# Autodesk Inventor assembly: サイクロイド減速機
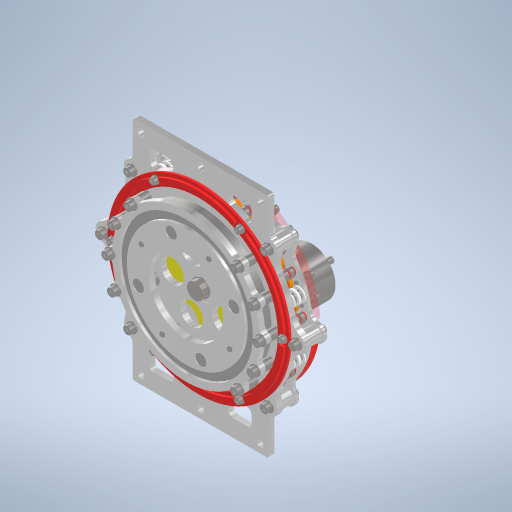
[picture p0: Inventor's stored thumbnail of the model, 512x512]
Saved by Autodesk Inventor 2024 (Build 280153000, 153)
## iProperties
Created: 2023-05-29
Part Number: サイクロイド減速機
Document SubType Name: Assembly
Designer: yuta2
Mass: 2238.9 g
Surface Area: 3502.49 cm^2
Volume: 607.759 cm^3
Density: 3.68387 g/cm^3
Author: yuta2
## Documents named in this file (32)
- C:\Users\yuta2\Documents\Inventor\CycloidDrive\サイクロイド減速機_大型\サイクロイド減速機.iam
- C:\Users\yuta2\Documents\Inventor\CycloidDrive\サイクロイド減速機_大型\サイクロイド減速機パラメータ.ipt
- C:\Users\yuta2\Documents\Inventor\CycloidDrive\サイクロイド減速機_大型\サイクロイドギア.ipt
- C:\Users\yuta2\Documents\Inventor\CycloidDrive\サイクロイド減速機_大型\ベース板_出力側.ipt
- C:\Users\yuta2\Documents\Inventor\CycloidDrive\サイクロイド減速機_大型\偏心軸ユニット.iam
- C:\Users\yuta2\Documents\Inventor\CycloidDrive\サイクロイド減速機_大型\出力板ユニット.iam
- C:\Users\yuta2\Documents\Inventor\CycloidDrive\サイクロイド減速機_大型\入力軸.ipt
- C:\Users\yuta2\Documents\Inventor\CycloidDrive\サイクロイド減速機_大型\出力ベアリング抑え.ipt
- C:\Users\yuta2\Documents\Inventor\CycloidDrive\サイクロイド減速機_大型\サイクロイド減速機\デザイン アクセラレータ\ボルト締結1.iam
- C:\Users\yuta2\Documents\Inventor\CycloidDrive\サイクロイド減速機_大型\外周ピンユニット.iam
- C:\Users\yuta2\Documents\Inventor\CycloidDrive\サイクロイド減速機_大型\ベース板入力側.ipt
- C:\Users\yuta2\Documents\Inventor\CycloidDrive\ベアリング\SMF148ZZ.ipt
- C:\Users\yuta2\Documents\Inventor\CycloidDrive\サイクロイド減速機_大型\RZ735.ipt
- C:\Users\yuta2\Documents\Inventor\CycloidDrive\サイクロイド減速機_大型\サイクロイド減速機\デザイン アクセラレータ\平歯車1.iam
- C:\Users\yuta2\Documents\Inventor\CycloidDrive\サイクロイド減速機_大型\サイクロイド減速機\デザイン アクセラレータ\平歯車2.iam
- C:\Users\yuta2\Documents\Inventor\CycloidDrive\サイクロイド減速機_大型\モーターマウント板.ipt
- C:\Users\yuta2\Documents\Inventor\CycloidDrive\サイクロイド減速機_大型\モーターマウント板固定部品.ipt
- C:\Users\yuta2\Documents\Inventor\CycloidDrive\サイクロイド減速機_大型\モーターマウント板固定部品2.ipt
- C:\Users\yuta2\Documents\Inventor\CycloidDrive\共通部品\インサートナットM4.ipt
- C:\Users\yuta2\Documents\Inventor\CycloidDrive\サイクロイド減速機_大型\サイクロイド減速機\デザイン アクセラレータ\ボルト締結2.iam
- C:\Users\yuta2\Documents\Inventor\CycloidDrive\サイクロイド減速機_大型\サイクロイド減速機\デザイン アクセラレータ\ボルト締結3.iam
- C:\Users\yuta2\Documents\Inventor\CycloidDrive\サイクロイド減速機_大型\外周ピン抑え.ipt
- C:\Users\yuta2\Documents\Inventor\CycloidDrive\サイクロイド減速機_大型\サイクロイド減速機\デザイン アクセラレータ\ボルト締結4.iam
- C:\Users\yuta2\Documents\Inventor\CycloidDrive\サイクロイド減速機_大型\ベース板連結棒.ipt
- C:\Users\yuta2\Documents\Inventor\CycloidDrive\サイクロイド減速機_大型\サイクロイド減速機\デザイン アクセラレータ\ボルト締結5.iam
- C:\Users\yuta2\Documents\Inventor\CycloidDrive\サイクロイド減速機_大型\出力ベアリング固定スペーサ.ipt
- C:\Users\yuta2\Documents\Inventor\CycloidDrive\サイクロイド減速機_大型\セットカラーSSCCJ8-5.ipt
- C:\Users\yuta2\Documents\Inventor\CycloidDrive\サイクロイド減速機_大型\ギアスペーサ1.ipt
- C:\Users\yuta2\Documents\Inventor\CycloidDrive\サイクロイド減速機_大型\ギアスペーサ2.ipt
- C:\Users\yuta2\Documents\Inventor\CycloidDrive\サイクロイド減速機_大型\外周ベアリングスペーサ1.ipt
- C:\Users\yuta2\Documents\Inventor\CycloidDrive\サイクロイド減速機_大型\外周ベアリングスペーサ.ipt
- C:\Users\yuta2\Documents\Inventor\CycloidDrive\サイクロイド減速機_大型\入力駆動ギアスペーサ.ipt
## Components (185 placed, 26 different names)
1. サイクロイド減速機パラメータ:1
2. サイクロイドギア:1 — 回転:1, 正接:5
3. ベース板_出力側:1 — 回転:3, 回転:9, 回転:25, 回転:26, 回転:30, メイト:18, メイト:19
4. 偏心軸ユニット:1 [sub-assembly] — 回転:1, 回転:2, 回転:5, 回転:10
5. サイクロイドギア:2 — 回転:2, 正接:2, 正接:4
6. 出力板ユニット:1 [sub-assembly] — 回転:3, 回転:5, 回転:6, 回転:32, 正接:4, 正接:5
7. 入力軸:1 — 回転:33, 回転:36, 回転:37
8. 出力ベアリング抑え:1 — 回転:6, メイト:15, メイト:16, 回転:29
9. ボルト締結:1 [sub-assembly] — メイト:15, メイト:16
10. ベース板入力側:1 — 円柱状:1, 回転:10, 回転:13, 回転:17, 回転:24, メイト:6, 回転:27, 回転:34, メイト:17
11. RZ735:1 — 回転:14, 回転:15, 回転:16
12. 平歯車:1 [sub-assembly] — 回転:13, 回転:47
13. 平歯車:2 [sub-assembly] — 回転:14
14. モーターマウント板:1 — 回転:15, 回転:16, 回転:18, 回転:19, 回転:20, 回転:21, メイト:13, メイト:14, 回転:35
15. モーターマウント板固定部品:1 — 回転:17, 回転:18, 回転:19, 回転:22, 回転:24, メイト:5
16. モーターマウント板固定部品2:1 — 回転:20, 回転:21, 回転:23
17. ボルト締結:2 [sub-assembly] — メイト:13, メイト:14
18. ボルト締結:3 [sub-assembly] — メイト:5, メイト:6
19. 外周ピン抑え:1 — 回転:25, 回転:26, メイト:7, メイト:8
20. SMF148ZZ:2 — 回転:35
21. SMF148ZZ:3 — 回転:32, 回転:33
22. SMF148ZZ:4 — 回転:34
23. セットカラーSSCCJ8-5:1 — 回転:36
24. セットカラーSSCCJ8-5:2 — 回転:37
25. 入力駆動ギアスペーサ:1 — 回転:47
26. 外周ピンユニット:1 [sub-assembly] — 回転:9, 円柱状:1
27. 外周ピンユニット:2 [sub-assembly]
28. 外周ピンユニット:3 [sub-assembly]
29. 外周ピンユニット:4 [sub-assembly]
30. 外周ピンユニット:5 [sub-assembly]
31. 外周ピンユニット:6 [sub-assembly]
32. 外周ピンユニット:7 [sub-assembly]
33. 外周ピンユニット:8 [sub-assembly]
34. 外周ピンユニット:9 [sub-assembly]
35. 外周ピンユニット:10 [sub-assembly] — 正接:2
36. 外周ピンユニット:11 [sub-assembly]
37. 外周ピンユニット:12 [sub-assembly]
38. 外周ピンユニット:13 [sub-assembly]
39. 外周ピンユニット:14 [sub-assembly]
40. 外周ピンユニット:15 [sub-assembly]
41. 外周ピンユニット:16 [sub-assembly]
42. 外周ピンユニット:17 [sub-assembly]
43. 外周ピンユニット:18 [sub-assembly]
44. 外周ピンユニット:19 [sub-assembly]
45. 外周ピンユニット:20 [sub-assembly]
46. 外周ピンユニット:21 [sub-assembly]
47. 外周ピンユニット:22 [sub-assembly] — メイト:17, 回転:38, 回転:39, 回転:40
48. 外周ピンユニット:23 [sub-assembly]
49. 外周ピンユニット:24 [sub-assembly]
50. 外周ピンユニット:25 [sub-assembly]
51. 外周ピンユニット:26 [sub-assembly] — 回転:42, 回転:43, 回転:46
52. 外周ピンユニット:27 [sub-assembly] — 回転:41, 回転:44, 回転:45
53. 外周ピンユニット:28 [sub-assembly]
54. 外周ピンユニット:29 [sub-assembly]
55. 外周ピンユニット:30 [sub-assembly]
56. インサートナットM4:1 — 回転:22
57. インサートナットM4:3
58. インサートナットM4:4
59. インサートナットM4:5
60. インサートナットM4:6
61. インサートナットM4:7
62. インサートナットM4:2 — 回転:23
63. インサートナットM4:8
64. インサートナットM4:9
65. インサートナットM4:10
66. インサートナットM4:11
67. インサートナットM4:12
68. ボルト締結:4 [sub-assembly] — メイト:7, メイト:8
69. ボルト締結:5 [sub-assembly]
70. ボルト締結:6 [sub-assembly]
71. ボルト締結:7 [sub-assembly]
72. ボルト締結:8 [sub-assembly]
73. ボルト締結:9 [sub-assembly]
74. 外周ベアリングスペーサ1:4 — 回転:44
75. 外周ベアリングスペーサ:1 — 回転:45
76. 外周ベアリングスペーサ1:1 — 回転:41
77. 外周ベアリングスペーサ1:3 — 回転:43
78. 外周ベアリングスペーサ:2 — 回転:46
79. 外周ベアリングスペーサ1:2 — 回転:42
80. ギアスペーサ1:2 — 回転:39
81. ギアスペーサ2:1 — 回転:40
82. ギアスペーサ1:1 — 回転:38
83. 外周ベアリングスペーサ1:5
84. 外周ベアリングスペーサ:3
85. 外周ベアリングスペーサ1:6
86. 外周ベアリングスペーサ1:7
87. 外周ベアリングスペーサ:4
88. 外周ベアリングスペーサ1:8
89. ギアスペーサ1:3
90. ギアスペーサ2:2
91. ギアスペーサ1:4
92. 外周ベアリングスペーサ1:9
93. 外周ベアリングスペーサ:5
94. 外周ベアリングスペーサ1:10
95. 外周ベアリングスペーサ1:11
96. 外周ベアリングスペーサ:6
97. 外周ベアリングスペーサ1:12
98. ギアスペーサ1:5
99. ギアスペーサ2:3
100. ギアスペーサ1:6
101. 外周ベアリングスペーサ1:13
102. 外周ベアリングスペーサ:7
103. 外周ベアリングスペーサ1:14
104. 外周ベアリングスペーサ1:15
105. 外周ベアリングスペーサ:8
106. 外周ベアリングスペーサ1:16
107. ギアスペーサ1:7
108. ギアスペーサ2:4
109. ギアスペーサ1:8
110. 外周ベアリングスペーサ1:17
111. 外周ベアリングスペーサ:9
112. 外周ベアリングスペーサ1:18
113. 外周ベアリングスペーサ1:19
114. 外周ベアリングスペーサ:10
115. 外周ベアリングスペーサ1:20
116. ギアスペーサ1:9
117. ギアスペーサ2:5
118. ギアスペーサ1:10
119. 外周ベアリングスペーサ1:21
120. 外周ベアリングスペーサ:11
121. 外周ベアリングスペーサ1:22
122. 外周ベアリングスペーサ1:23
123. 外周ベアリングスペーサ:12
124. 外周ベアリングスペーサ1:24
125. ギアスペーサ1:11
126. ギアスペーサ2:6
127. ギアスペーサ1:12
128. 外周ベアリングスペーサ1:25
129. 外周ベアリングスペーサ:13
130. 外周ベアリングスペーサ1:26
131. 外周ベアリングスペーサ1:27
132. 外周ベアリングスペーサ:14
133. 外周ベアリングスペーサ1:28
134. ギアスペーサ1:13
135. ギアスペーサ2:7
136. ギアスペーサ1:14
137. 外周ベアリングスペーサ1:29
138. 外周ベアリングスペーサ:15
139. 外周ベアリングスペーサ1:30
140. 外周ベアリングスペーサ1:31
141. 外周ベアリングスペーサ:16
142. 外周ベアリングスペーサ1:32
143. ギアスペーサ1:15
144. ギアスペーサ2:8
145. ギアスペーサ1:16
146. 外周ベアリングスペーサ1:33
147. 外周ベアリングスペーサ:17
148. 外周ベアリングスペーサ1:34
149. 外周ベアリングスペーサ1:35
150. 外周ベアリングスペーサ:18
151. 外周ベアリングスペーサ1:36
152. ギアスペーサ1:17
153. ギアスペーサ2:9
154. ギアスペーサ1:18
155. 外周ベアリングスペーサ1:37
156. 外周ベアリングスペーサ:19
157. 外周ベアリングスペーサ1:38
158. 外周ベアリングスペーサ1:39
159. 外周ベアリングスペーサ:20
160. 外周ベアリングスペーサ1:40
161. ギアスペーサ1:19
162. ギアスペーサ2:10
163. ギアスペーサ1:20
164. ベース板連結棒:1 — 回転:27
165. ベース板連結棒:2
166. ベース板連結棒:3
167. ベース板連結棒:4
168. ベース板連結棒:5
169. ベース板連結棒:6
170. ボルト締結:10 [sub-assembly] — メイト:18, メイト:19
171. ボルト締結:11 [sub-assembly]
172. ボルト締結:12 [sub-assembly]
173. ボルト締結:13 [sub-assembly]
174. ボルト締結:14 [sub-assembly]
175. ボルト締結:15 [sub-assembly]
176. 出力ベアリング固定スペーサ:1 — 回転:29, 回転:30
177. 出力ベアリング固定スペーサ:2
178. 出力ベアリング固定スペーサ:3
179. 出力ベアリング固定スペーサ:4
180. 出力ベアリング固定スペーサ:5
181. 出力ベアリング固定スペーサ:6
182. 出力ベアリング固定スペーサ:7
183. 出力ベアリング固定スペーサ:8
184. 出力ベアリング固定スペーサ:9
185. 出力ベアリング固定スペーサ:10
## Component patterns: (30 elements, first: 外周ピンユニット:1), (6 elements, first: インサートナットM4:1), (6 elements, first: インサートナットM4:2), (6 elements, first: ボルト締結:4), (2 elements), (3 elements), (2 elements), (10 elements, first: 外周ベアリングスペーサ1:4 + 外周ベアリングスペーサ:1 + 外周ベアリングスペーサ1:1 + 外周ベアリングスペーサ1:3 + 外周ベアリングスペーサ:2 + 外周ベアリングスペーサ1:2 + ギアスペーサ1:2 + ギアスペーサ2:1 + ギアスペーサ1:1), (3 elements, first: ベース板連結棒:1), コンポーネント パターン 7:2 (3 elements), (2 elements, first: ボルト締結:10), コンポーネント パターン 9:2 (2 elements), コンポーネント パターン 9:3 (2 elements), (5 elements, first: 出力ベアリング固定スペーサ:1), コンポーネント パターン 11:2 (5 elements)
## Relationships (55: RevoluteJoint 40, Mate 11, Tangent 3, CylindricalJoint 1)
- 回転:1 [RevoluteJoint]: サイクロイドギア:1 ↔ 偏心軸ユニット:1
- 回転:2 [RevoluteJoint]: 偏心軸ユニット:1 ↔ サイクロイドギア:2
- 回転:3 [RevoluteJoint]: ベース板_出力側:1 ↔ 出力板ユニット:1
- 回転:5 [RevoluteJoint] (0.5 mm): 偏心軸ユニット:1 ↔ 出力板ユニット:1
- 回転:6 [RevoluteJoint]: 出力板ユニット:1 ↔ 出力ベアリング抑え:1
- 回転:9 [RevoluteJoint]: ベース板_出力側:1 ↔ 外周ピンユニット:1
- 円柱状:1 [CylindricalJoint]: ベース板入力側:1 ↔ 外周ピンユニット:1
- 回転:10 [RevoluteJoint] (-0.5 mm): 偏心軸ユニット:1 ↔ ベース板入力側:1
- 回転:13 [RevoluteJoint] (1 mm): ベース板入力側:1 ↔ 平歯車:1
- 回転:14 [RevoluteJoint] (0.5 mm): RZ735:1 ↔ 平歯車:2
- 回転:15 [RevoluteJoint]: RZ735:1 ↔ モーターマウント板:1
- 回転:16 [RevoluteJoint]: RZ735:1 ↔ モーターマウント板:1
- 回転:17 [RevoluteJoint]: ベース板入力側:1 ↔ モーターマウント板固定部品:1
- 回転:18 [RevoluteJoint]: モーターマウント板:1 ↔ モーターマウント板固定部品:1
- 回転:19 [RevoluteJoint]: モーターマウント板:1 ↔ モーターマウント板固定部品:1
- 回転:20 [RevoluteJoint]: モーターマウント板:1 ↔ モーターマウント板固定部品2:1
- 回転:21 [RevoluteJoint]: モーターマウント板:1 ↔ モーターマウント板固定部品2:1
- 回転:22 [RevoluteJoint]: モーターマウント板固定部品:1 ↔ インサートナットM4:1
- 回転:23 [RevoluteJoint]: モーターマウント板固定部品2:1 ↔ インサートナットM4:2
- 回転:24 [RevoluteJoint]: ベース板入力側:1 ↔ モーターマウント板固定部品:1
- メイト:5 [Mate]: モーターマウント板固定部品:1 ↔ ボルト締結:3
- メイト:6 [Mate]: ベース板入力側:1 ↔ ボルト締結:3
- 回転:25 [RevoluteJoint]: ベース板_出力側:1 ↔ 外周ピン抑え:1
- 回転:26 [RevoluteJoint]: ベース板_出力側:1 ↔ 外周ピン抑え:1
- メイト:7 [Mate]: 外周ピン抑え:1 ↔ ボルト締結:4
- メイト:8 [Mate]: 外周ピン抑え:1 ↔ ボルト締結:4
- 回転:27 [RevoluteJoint]: ベース板入力側:1 ↔ ベース板連結棒:1
- メイト:13 [Mate]: モーターマウント板:1 ↔ ボルト締結:2
- メイト:14 [Mate]: モーターマウント板:1 ↔ ボルト締結:2
- メイト:15 [Mate]: 出力ベアリング抑え:1 ↔ ボルト締結:1
- メイト:16 [Mate]: 出力ベアリング抑え:1 ↔ ボルト締結:1
- 回転:29 [RevoluteJoint]: 出力ベアリング抑え:1 ↔ 出力ベアリング固定スペーサ:1
- 回転:30 [RevoluteJoint]: ベース板_出力側:1 ↔ 出力ベアリング固定スペーサ:1
- 回転:32 [RevoluteJoint]: 出力板ユニット:1 ↔ SMF148ZZ:3
- 回転:33 [RevoluteJoint] (5 mm): 入力軸:1 ↔ SMF148ZZ:3
- 回転:34 [RevoluteJoint]: ベース板入力側:1 ↔ SMF148ZZ:4
- 回転:35 [RevoluteJoint]: モーターマウント板:1 ↔ SMF148ZZ:2
- メイト:17 [Mate]: ベース板入力側:1 ↔ 外周ピンユニット:22
- 正接:2 [Tangent]: サイクロイドギア:2 ↔ 外周ピンユニット:10
- 正接:4 [Tangent]: サイクロイドギア:2 ↔ 出力板ユニット:1
- 正接:5 [Tangent]: サイクロイドギア:1 ↔ 出力板ユニット:1
- 回転:36 [RevoluteJoint]: 入力軸:1 ↔ セットカラーSSCCJ8-5:1
- 回転:37 [RevoluteJoint]: 入力軸:1 ↔ セットカラーSSCCJ8-5:2
- メイト:18 [Mate]: ベース板_出力側:1 ↔ ボルト締結:10
- メイト:19 [Mate]: ベース板_出力側:1 ↔ ボルト締結:10
- 回転:38 [RevoluteJoint]: 外周ピンユニット:22 ↔ ギアスペーサ1:1
- 回転:39 [RevoluteJoint]: 外周ピンユニット:22 ↔ ギアスペーサ1:2
- 回転:40 [RevoluteJoint]: 外周ピンユニット:22 ↔ ギアスペーサ2:1
- 回転:41 [RevoluteJoint]: 外周ピンユニット:27 ↔ 外周ベアリングスペーサ1:1
- 回転:42 [RevoluteJoint]: 外周ピンユニット:26 ↔ 外周ベアリングスペーサ1:2
- 回転:43 [RevoluteJoint]: 外周ピンユニット:26 ↔ 外周ベアリングスペーサ1:3
- 回転:44 [RevoluteJoint]: 外周ピンユニット:27 ↔ 外周ベアリングスペーサ1:4
- 回転:45 [RevoluteJoint]: 外周ピンユニット:27 ↔ 外周ベアリングスペーサ:1
- 回転:46 [RevoluteJoint]: 外周ピンユニット:26 ↔ 外周ベアリングスペーサ:2
- 回転:47 [RevoluteJoint]: 平歯車:1 ↔ 入力駆動ギアスペーサ:1
## Named parameters: N_pin = 30, r = 2 mm, D = 150 mm, Dc = 4.83871 mm, D_pin = 8 mm
